# Autodesk Inventor assembly: Assy_hand
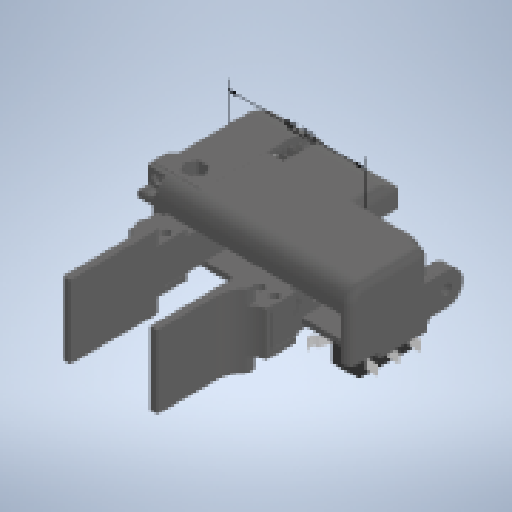
[picture p0: Inventor's stored thumbnail of the model, 512x512]
Saved by Autodesk Inventor 2024.1 (Build 281209000, 209)
## iProperties
Created: 2025-02-23
Part Number: Assy_hand
Document SubType Name: Assembly
Designer: hibik
Author: hibik
## Documents named in this file (11)
- C:\Users\hibik\Documents\Robomech\RESCUE\ORCA\hard\arm\Assy_hand.iam
- C:\Users\hibik\Documents\Robomech\RESCUE\ORCA\hard\arm\hand_motor_setter_base.ipt
- C:\Users\hibik\Documents\Robomech\RESCUE\ORCA\hard\arm\hand_motor_setter_cover_under.ipt
- C:\Users\hibik\Documents\Robomech\RESCUE\ORCA\hard\std_parts\motor_M4_55.ipt
- C:\Users\hibik\Documents\Robomech\RESCUE\ORCA\hard\arm\hand_finger_inside.ipt
- C:\Users\hibik\Documents\Robomech\RESCUE\ORCA\hard\arm\hand_finger_outside.ipt
- C:\Users\hibik\Documents\Robomech\RESCUE\ORCA\hard\std_parts\limit_switch.ipt
- C:\Users\hibik\Documents\Robomech\RESCUE\ORCA\hard\arm\hand_finger.ipt
- C:\Users\hibik\Documents\Robomech\RESCUE\ORCA\hard\arm\hand_gear_hand.ipt
- C:\Users\hibik\Documents\Robomech\RESCUE\ORCA\hard\std_parts\bearing_6_10_3.ipt
- C:\Users\hibik\Documents\Robomech\RESCUE\ORCA\hard\arm\hand_finger_cover.ipt
## Components (13 placed, 10 different names)
1. hand_motor_setter_base:1 — 挿入:1, 挿入:2, 挿入:3, 角度:1, 挿入:5, 挿入:6, フラッシュ:2, フラッシュ:3, 挿入:7, 挿入:8, 挿入:11, 挿入:12, 角度:2, 角度:3, 対称度:1, 角度:4
2. hand_motor_setter_cover_under:1 — 挿入:1, 挿入:2, 挿入:13, メイト:1, フラッシュ:5, フラッシュ:6, 挿入:14
3. motor_M4_55:1 — 挿入:3, 角度:1
4. hand_finger_inside:1 — 挿入:4, フラッシュ:3, フラッシュ:4, 挿入:9, 挿入:10
5. hand_finger_outside:1 — 挿入:4, フラッシュ:2, フラッシュ:4
6. limit_switch:1 — 挿入:5, 挿入:6
7. hand_finger:1 — 挿入:7, 挿入:8
8. hand_finger:2 — 挿入:9, 挿入:10
9. hand_gear_hand:1 — 挿入:11, 角度:2
10. bearing_6_10_3:1 — 挿入:12
11. bearing_6_10_3:2 — 挿入:13, メイト:2
12. limit_switch:2 — メイト:1, フラッシュ:5, フラッシュ:6
13. hand_finger_cover:1 — 角度:3, 対称度:1, 挿入:14
## Relationships (27: Insert 14, Flush 6, Angle 4, Mate 2, Symmetry 1)
- 挿入:1 [Insert]: hand_motor_setter_base:1 ↔ hand_motor_setter_cover_under:1
- 挿入:2 [Insert]: hand_motor_setter_base:1 ↔ hand_motor_setter_cover_under:1
- 挿入:3 [Insert]: hand_motor_setter_base:1 ↔ motor_M4_55:1
- 角度:1 [Angle] (0 deg): hand_motor_setter_base:1 ↔ motor_M4_55:1
- 挿入:4 [Insert]: hand_finger_inside:1 ↔ hand_finger_outside:1
- 挿入:5 [Insert]: hand_motor_setter_base:1 ↔ limit_switch:1
- 挿入:6 [Insert]: hand_motor_setter_base:1 ↔ limit_switch:1
- フラッシュ:2 [Flush]: hand_motor_setter_base:1 ↔ hand_finger_outside:1
- フラッシュ:3 [Flush]: hand_motor_setter_base:1 ↔ hand_finger_inside:1
- フラッシュ:4 [Flush]: hand_finger_inside:1 ↔ hand_finger_outside:1
- 挿入:7 [Insert]: hand_motor_setter_base:1 ↔ hand_finger:1
- 挿入:8 [Insert]: hand_motor_setter_base:1 ↔ hand_finger:1
- 挿入:9 [Insert]: hand_finger_inside:1 ↔ hand_finger:2
- 挿入:10 [Insert]: hand_finger_inside:1 ↔ hand_finger:2
- 挿入:11 [Insert] (6 mm): hand_motor_setter_base:1 ↔ hand_gear_hand:1
- 挿入:12 [Insert]: hand_motor_setter_base:1 ↔ bearing_6_10_3:1
- 挿入:13 [Insert]: hand_motor_setter_cover_under:1 ↔ bearing_6_10_3:2
- 角度:2 [Angle] (30 deg): hand_motor_setter_base:1 ↔ hand_gear_hand:1
- メイト:1 [Mate] (3 mm): hand_motor_setter_cover_under:1 ↔ limit_switch:2
- フラッシュ:5 [Flush]: hand_motor_setter_cover_under:1 ↔ limit_switch:2
- フラッシュ:6 [Flush] (3 mm): hand_motor_setter_cover_under:1 ↔ limit_switch:2
- 角度:3 [Angle] (0 deg): hand_motor_setter_base:1 ↔ hand_finger_cover:1
- メイト:2 [Mate]: bearing_6_10_3:2
- 対称度:1 [Symmetry]: hand_motor_setter_base:1 ↔ hand_finger_cover:1
- フラッシュ:7 [Flush]
- 角度:4 [Angle] (0 deg): hand_motor_setter_base:1
- 挿入:14 [Insert]: hand_motor_setter_cover_under:1 ↔ hand_finger_cover:1
